# Autodesk Inventor assembly: MaquinaDeCorte
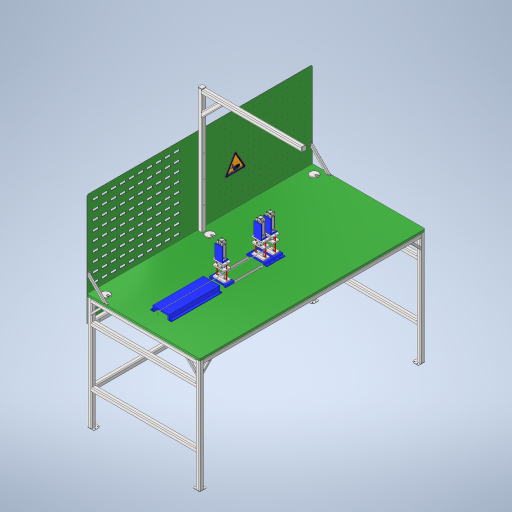
[picture p0: Inventor's stored thumbnail of the model, 512x512]
Saved by Autodesk Inventor 2023 (Build 270158000, 158)
## iProperties
Created: 2023-04-07
Part Number: MaquinaDeCorte
Document SubType Name: Assembly
Designer: Lenovo
Author: Lenovo
## Documents named in this file (35)
- D:\Esdek\Gemelo Digital\Corte de Tubos\MaquinaDeCorte.iam
- D:\Esdek\Gemelo Digital\Corte de Tubos\CADimportados\PistónElectromecánico\1470706 EPCO-25-300-3P-ST-E---(0).iam
- D:\Esdek\Gemelo Digital\Corte de Tubos\SoporteElectromecánico.ipt
- D:\Esdek\Gemelo Digital\Corte de Tubos\CADimportados\Main Table Assembly.ipt
- D:\Esdek\Gemelo Digital\Corte de Tubos\CADimportados\PistónHidráulico\163321 DNC-32-50-PPV---(asm_0).iam
- D:\Esdek\Gemelo Digital\Corte de Tubos\SoporteHidráhulicos.ipt
- D:\Esdek\Gemelo Digital\Corte de Tubos\PlacaSuperiorHidráulicos.ipt
- D:\Esdek\Gemelo Digital\Corte de Tubos\CodoHidráulicos.ipt
- D:\Esdek\Gemelo Digital\Corte de Tubos\PlacaMediaHidráulicos.ipt
- D:\Esdek\Gemelo Digital\Corte de Tubos\Cuchilla.ipt
- D:\Esdek\Gemelo Digital\Corte de Tubos\PlacaBaseHidráulicos.ipt
- D:\Esdek\Gemelo Digital\Corte de Tubos\BaseCuchilla.ipt
- D:\Esdek\Gemelo Digital\Corte de Tubos\CADimportados\Knutec.de - Warning, Crushing of hands, according ISO EN DIN 7010_200.ipt
- D:\Esdek\Gemelo Digital\Corte de Tubos\CADimportados\PistónHidráulico\163321 DNC-32-50-PPV---(asm_0)_CPY.iam
- D:\Esdek\Gemelo Digital\Corte de Tubos\SoporteHidráhulicos_CPY.ipt
- D:\Esdek\Gemelo Digital\Corte de Tubos\PlacaSuperiorHidráulicos_CPY.ipt
- D:\Esdek\Gemelo Digital\Corte de Tubos\CodoHidráulicos_CPY.ipt
- D:\Esdek\Gemelo Digital\Corte de Tubos\PlacaMediaHidráulicos_CPY.ipt
- D:\Esdek\Gemelo Digital\Corte de Tubos\PlacaBaseHidráulicos_CPY.ipt
- D:\Esdek\Gemelo Digital\Corte de Tubos\SoporteTubosInferior.ipt
- D:\Esdek\Gemelo Digital\Corte de Tubos\SoporteTubosSuperior.ipt
- D:\Esdek\Gemelo Digital\Corte de Tubos\CADimportados\PistónHidráulico\163321 DNC-32-50-PPV---(asm_0)_CPY_CPY.iam
- D:\Esdek\Gemelo Digital\Corte de Tubos\SoporteHidráhulicos_CPY_CPY.ipt
- D:\Esdek\Gemelo Digital\Corte de Tubos\PlacaSuperiorHidráulicos_CPY_CPY.ipt
- D:\Esdek\Gemelo Digital\Corte de Tubos\CodoHidráulicos_CPY_CPY.ipt
- D:\Esdek\Gemelo Digital\Corte de Tubos\PlacaMediaHidráulicos_CPY_CPY.ipt
- D:\Esdek\Gemelo Digital\Corte de Tubos\PlacaBaseHidráulicos_CPY_CPY.ipt
- D:\Esdek\Gemelo Digital\Corte de Tubos\SoporteTubosInferior_CPY.ipt
- D:\Esdek\Gemelo Digital\Corte de Tubos\SoporteTubosSuperior_CPY.ipt
- D:\Esdek\Gemelo Digital\Corte de Tubos\AcopleActuadorCarro.ipt
- D:\Esdek\Gemelo Digital\Corte de Tubos\CarroSuperior.ipt
- D:\Esdek\Gemelo Digital\Corte de Tubos\CarroFijoSuperior.ipt
- D:\Esdek\Gemelo Digital\Corte de Tubos\Sujetador.ipt
- D:\Esdek\Gemelo Digital\Corte de Tubos\SoporteMaterial.ipt
- D:\Esdek\Gemelo Digital\Corte de Tubos\Material.ipt
## Components (41 placed, 34 different names)
1. 1470706 EPCO-25-300-3P-ST-E---(0):1 [sub-assembly] — Mate:30, Mate:31, Mate:32, Mate:33, Mate:34
2. Main Table Assembly:1 — Mate:25, Angle:1, Mate:26, Mate:27, Mate:28, Mate:29, Mate:87, Mate:88, Mate:89, Mate:93, Mate:94, Mate:95, Mate:111, Mate:112, Mate:113
3. 163321 DNC-32-50-PPV---(asm_0):1 [sub-assembly] — Mate:4, Mate:5, Mate:6, Mate:12
4. SoporteHidráhulicos:1 — Mate:4, Mate:5, Mate:6, Mate:7, Mate:8, Mate:9
5. PlacaSuperiorHidráulicos:1 — Mate:7, Mate:8, Mate:9, Mate:10, Mate:11, Mate:24, Mate:107, Mate:108, Mate:109, Mate:110
6. CodoHidráulicos:1 — Mate:10, Mate:11, Mate:12, Mate:13, Mate:14, Mate:15
7. PlacaMediaHidráulicos:1 — Mate:13, Mate:14, Mate:15, Mate:16, Mate:17, Mate:18, Mate:22, Mate:23
8. Cuchilla:1 — Mate:16, Mate:17, Mate:18
9. PlacaBaseHidráulicos:1 — Mate:19, Mate:20, Mate:21, Mate:22, Mate:23, Mate:96, Mate:97, Mate:98
10. BaseCuchilla:1 — Mate:19, Mate:20, Mate:21, Mate:24, Mate:115
11. Knutec.de - Warning, Crushing of hands, according ISO EN DIN 7010_200:1 — Mate:25, Angle:1, Mate:26
12. SoporteElectromecánico:1 — Mate:27, Mate:28, Mate:29, Mate:30, Mate:31, Mate:32, Angle:2
13. CodoHidráulicos:2 — Mate:33, Mate:34, Angle:2, Mate:78, Mate:79, Mate:80
14. 163321 DNC-32-50-PPV---(asm_0)_CPY:1 [sub-assembly] — Mate:36, Mate:37, Mate:38, Mate:42
15. SoporteHidráhulicos_CPY:1 — Mate:36, Mate:37, Mate:38, Mate:39, Mate:40, Mate:41
16. PlacaSuperiorHidráulicos_CPY:1 — Mate:39, Mate:40, Mate:41, Mate:43, Mate:44, Mate:50, Mate:104, Mate:105, Mate:106
17. CodoHidráulicos_CPY:1 — Mate:42, Mate:43, Mate:44, Mate:45, Mate:46, Mate:47
18. PlacaMediaHidráulicos_CPY:1 — Mate:45, Mate:46, Mate:47, Mate:48, Mate:49, Mate:54, Mate:55, Mate:56, Mate:103
19. PlacaBaseHidráulicos_CPY:1 — Mate:48, Mate:49, Mate:50, Mate:51, Mate:52, Mate:53, Mate:90, Mate:91, Mate:92
20. SoporteTubosInferior:1 — Mate:51, Mate:52, Mate:53
21. SoporteTubosSuperior:1 — Mate:54, Mate:55, Mate:56
22. 163321 DNC-32-50-PPV---(asm_0)_CPY_CPY:1 [sub-assembly] — Mate:57, Mate:58, Mate:59, Mate:65
23. SoporteHidráhulicos_CPY_CPY:1 — Mate:57, Mate:58, Mate:59, Mate:60, Mate:61, Mate:62
24. PlacaSuperiorHidráulicos_CPY_CPY:1 — Mate:60, Mate:61, Mate:62, Mate:63, Mate:64, Mate:69, Mate:99, Mate:100, Mate:102
25. CodoHidráulicos_CPY_CPY:1 — Mate:63, Mate:64, Mate:65, Mate:66, Mate:67, Mate:68
26. PlacaMediaHidráulicos_CPY_CPY:1 — Mate:66, Mate:67, Mate:68, Mate:70, Mate:71, Mate:75, Mate:76, Mate:77, Mate:101
27. PlacaBaseHidráulicos_CPY_CPY:1 — Mate:69, Mate:70, Mate:71, Mate:72, Mate:73, Mate:74, Mate:84, Mate:85, Mate:86
28. SoporteTubosInferior_CPY:1 — Mate:72, Mate:73, Mate:74
29. SoporteTubosSuperior_CPY:1 — Mate:75, Mate:76, Mate:77
30. AcopleActuadorCarro:1 — Mate:78, Mate:79, Mate:80, Mate:81, Mate:82, Mate:83
31. CarroSuperior:1 — Mate:81, Mate:82, Mate:83, Mate:84, Mate:85, Mate:86
32. CarroFijoSuperior:1 — Mate:87, Mate:88, Mate:89, Mate:90, Mate:91, Mate:92
33. CarroFijoSuperior:2 — Mate:93, Mate:94, Mate:95, Mate:96, Mate:97, Mate:98
34. Sujetador:1 — Mate:99, Mate:100
35. Sujetador:2 — Mate:101, Mate:102
36. Sujetador:3 — Mate:103, Mate:104
37. Sujetador:4 — Mate:107, Mate:108
38. Sujetador:5 — Mate:109, Mate:110
39. Sujetador:6 — Mate:105, Mate:106
40. SoporteMaterial:1 — Mate:111, Mate:112, Mate:113, Mate:114
41. Material:1 — Mate:114, Mate:115
## Relationships (113: Mate 111, Angle 2)
- Mate:4: 163321 DNC-32-50-PPV---(asm_0):1 ↔ SoporteHidráhulicos:1
- Mate:5: 163321 DNC-32-50-PPV---(asm_0):1 ↔ SoporteHidráhulicos:1
- Mate:6: 163321 DNC-32-50-PPV---(asm_0):1 ↔ SoporteHidráhulicos:1
- Mate:7: SoporteHidráhulicos:1 ↔ PlacaSuperiorHidráulicos:1
- Mate:8: SoporteHidráhulicos:1 ↔ PlacaSuperiorHidráulicos:1
- Mate:9: SoporteHidráhulicos:1 ↔ PlacaSuperiorHidráulicos:1
- Mate:10: PlacaSuperiorHidráulicos:1 ↔ CodoHidráulicos:1
- Mate:11: PlacaSuperiorHidráulicos:1 ↔ CodoHidráulicos:1
- Mate:12: 163321 DNC-32-50-PPV---(asm_0):1 ↔ CodoHidráulicos:1
- Mate:13: CodoHidráulicos:1 ↔ PlacaMediaHidráulicos:1
- Mate:14: CodoHidráulicos:1 ↔ PlacaMediaHidráulicos:1
- Mate:15: CodoHidráulicos:1 ↔ PlacaMediaHidráulicos:1
- Mate:16: PlacaMediaHidráulicos:1 ↔ Cuchilla:1
- Mate:17: PlacaMediaHidráulicos:1 ↔ Cuchilla:1
- Mate:18: PlacaMediaHidráulicos:1 ↔ Cuchilla:1
- Mate:19: PlacaBaseHidráulicos:1 ↔ BaseCuchilla:1
- Mate:20: PlacaBaseHidráulicos:1 ↔ BaseCuchilla:1
- Mate:21: PlacaBaseHidráulicos:1 ↔ BaseCuchilla:1
- Mate:22: PlacaMediaHidráulicos:1 ↔ PlacaBaseHidráulicos:1
- Mate:23: PlacaMediaHidráulicos:1 ↔ PlacaBaseHidráulicos:1
- Mate:24 (115.5 mm): PlacaSuperiorHidráulicos:1 ↔ BaseCuchilla:1
- Mate:25: Main Table Assembly:1 ↔ Knutec.de - Warning, Crushing of hands, according ISO EN DIN 7010_200:1
- Angle:1 (180 deg): Main Table Assembly:1 ↔ Knutec.de - Warning, Crushing of hands, according ISO EN DIN 7010_200:1
- Mate:26: Main Table Assembly:1 ↔ Knutec.de - Warning, Crushing of hands, according ISO EN DIN 7010_200:1
- Mate:27: Main Table Assembly:1 ↔ SoporteElectromecánico:1
- Mate:28: Main Table Assembly:1 ↔ SoporteElectromecánico:1
- Mate:29: Main Table Assembly:1 ↔ SoporteElectromecánico:1
- Mate:30: 1470706 EPCO-25-300-3P-ST-E---(0):1 ↔ SoporteElectromecánico:1
- Mate:31: 1470706 EPCO-25-300-3P-ST-E---(0):1 ↔ SoporteElectromecánico:1
- Mate:32: 1470706 EPCO-25-300-3P-ST-E---(0):1 ↔ SoporteElectromecánico:1
- Mate:33: 1470706 EPCO-25-300-3P-ST-E---(0):1 ↔ CodoHidráulicos:2
- Mate:34: 1470706 EPCO-25-300-3P-ST-E---(0):1 ↔ CodoHidráulicos:2
- Angle:2 (0 deg): SoporteElectromecánico:1 ↔ CodoHidráulicos:2
- Mate:36: 163321 DNC-32-50-PPV---(asm_0)_CPY:1 ↔ SoporteHidráhulicos_CPY:1
- Mate:37: 163321 DNC-32-50-PPV---(asm_0)_CPY:1 ↔ SoporteHidráhulicos_CPY:1
- Mate:38: 163321 DNC-32-50-PPV---(asm_0)_CPY:1 ↔ SoporteHidráhulicos_CPY:1
- Mate:39: SoporteHidráhulicos_CPY:1 ↔ PlacaSuperiorHidráulicos_CPY:1
- Mate:40: SoporteHidráhulicos_CPY:1 ↔ PlacaSuperiorHidráulicos_CPY:1
- Mate:41: SoporteHidráhulicos_CPY:1 ↔ PlacaSuperiorHidráulicos_CPY:1
- Mate:42: 163321 DNC-32-50-PPV---(asm_0)_CPY:1 ↔ CodoHidráulicos_CPY:1
- Mate:43: PlacaSuperiorHidráulicos_CPY:1 ↔ CodoHidráulicos_CPY:1
- Mate:44: PlacaSuperiorHidráulicos_CPY:1 ↔ CodoHidráulicos_CPY:1
- Mate:45: CodoHidráulicos_CPY:1 ↔ PlacaMediaHidráulicos_CPY:1
- Mate:46: CodoHidráulicos_CPY:1 ↔ PlacaMediaHidráulicos_CPY:1
- Mate:47: CodoHidráulicos_CPY:1 ↔ PlacaMediaHidráulicos_CPY:1
- Mate:48: PlacaMediaHidráulicos_CPY:1 ↔ PlacaBaseHidráulicos_CPY:1
- Mate:49: PlacaMediaHidráulicos_CPY:1 ↔ PlacaBaseHidráulicos_CPY:1
- Mate:50 (125.5 mm): PlacaSuperiorHidráulicos_CPY:1 ↔ PlacaBaseHidráulicos_CPY:1
- Mate:51: PlacaBaseHidráulicos_CPY:1 ↔ SoporteTubosInferior:1
- Mate:52: PlacaBaseHidráulicos_CPY:1 ↔ SoporteTubosInferior:1
- Mate:53: PlacaBaseHidráulicos_CPY:1 ↔ SoporteTubosInferior:1
- Mate:54: PlacaMediaHidráulicos_CPY:1 ↔ SoporteTubosSuperior:1
- Mate:55: PlacaMediaHidráulicos_CPY:1 ↔ SoporteTubosSuperior:1
- Mate:56: PlacaMediaHidráulicos_CPY:1 ↔ SoporteTubosSuperior:1
- Mate:57: 163321 DNC-32-50-PPV---(asm_0)_CPY_CPY:1 ↔ SoporteHidráhulicos_CPY_CPY:1
- Mate:58: 163321 DNC-32-50-PPV---(asm_0)_CPY_CPY:1 ↔ SoporteHidráhulicos_CPY_CPY:1
- Mate:59: 163321 DNC-32-50-PPV---(asm_0)_CPY_CPY:1 ↔ SoporteHidráhulicos_CPY_CPY:1
- Mate:60: SoporteHidráhulicos_CPY_CPY:1 ↔ PlacaSuperiorHidráulicos_CPY_CPY:1
- Mate:61: SoporteHidráhulicos_CPY_CPY:1 ↔ PlacaSuperiorHidráulicos_CPY_CPY:1
- Mate:62: SoporteHidráhulicos_CPY_CPY:1 ↔ PlacaSuperiorHidráulicos_CPY_CPY:1
- Mate:63: PlacaSuperiorHidráulicos_CPY_CPY:1 ↔ CodoHidráulicos_CPY_CPY:1
- Mate:64: PlacaSuperiorHidráulicos_CPY_CPY:1 ↔ CodoHidráulicos_CPY_CPY:1
- Mate:65: 163321 DNC-32-50-PPV---(asm_0)_CPY_CPY:1 ↔ CodoHidráulicos_CPY_CPY:1
- Mate:66: CodoHidráulicos_CPY_CPY:1 ↔ PlacaMediaHidráulicos_CPY_CPY:1
- Mate:67: CodoHidráulicos_CPY_CPY:1 ↔ PlacaMediaHidráulicos_CPY_CPY:1
- Mate:68: CodoHidráulicos_CPY_CPY:1 ↔ PlacaMediaHidráulicos_CPY_CPY:1
- Mate:69 (125.5 mm): PlacaSuperiorHidráulicos_CPY_CPY:1 ↔ PlacaBaseHidráulicos_CPY_CPY:1
- Mate:70: PlacaMediaHidráulicos_CPY_CPY:1 ↔ PlacaBaseHidráulicos_CPY_CPY:1
- Mate:71: PlacaMediaHidráulicos_CPY_CPY:1 ↔ PlacaBaseHidráulicos_CPY_CPY:1
- Mate:72: PlacaBaseHidráulicos_CPY_CPY:1 ↔ SoporteTubosInferior_CPY:1
- Mate:73: PlacaBaseHidráulicos_CPY_CPY:1 ↔ SoporteTubosInferior_CPY:1
- Mate:74: PlacaBaseHidráulicos_CPY_CPY:1 ↔ SoporteTubosInferior_CPY:1
- Mate:75: PlacaMediaHidráulicos_CPY_CPY:1 ↔ SoporteTubosSuperior_CPY:1
- Mate:76: PlacaMediaHidráulicos_CPY_CPY:1 ↔ SoporteTubosSuperior_CPY:1
- Mate:77: PlacaMediaHidráulicos_CPY_CPY:1 ↔ SoporteTubosSuperior_CPY:1
- Mate:78: CodoHidráulicos:2 ↔ AcopleActuadorCarro:1
- Mate:79: CodoHidráulicos:2 ↔ AcopleActuadorCarro:1
- Mate:80: CodoHidráulicos:2 ↔ AcopleActuadorCarro:1
- Mate:81: AcopleActuadorCarro:1 ↔ CarroSuperior:1
- Mate:82: AcopleActuadorCarro:1 ↔ CarroSuperior:1
- Mate:83: AcopleActuadorCarro:1 ↔ CarroSuperior:1
- Mate:84: PlacaBaseHidráulicos_CPY_CPY:1 ↔ CarroSuperior:1
- Mate:85: PlacaBaseHidráulicos_CPY_CPY:1 ↔ CarroSuperior:1
- Mate:86: PlacaBaseHidráulicos_CPY_CPY:1 ↔ CarroSuperior:1
- Mate:87: Main Table Assembly:1 ↔ CarroFijoSuperior:1
- Mate:88: Main Table Assembly:1 ↔ CarroFijoSuperior:1
- Mate:89: Main Table Assembly:1 ↔ CarroFijoSuperior:1
- Mate:90: PlacaBaseHidráulicos_CPY:1 ↔ CarroFijoSuperior:1
- Mate:91: PlacaBaseHidráulicos_CPY:1 ↔ CarroFijoSuperior:1
- Mate:92: PlacaBaseHidráulicos_CPY:1 ↔ CarroFijoSuperior:1
- Mate:93: Main Table Assembly:1 ↔ CarroFijoSuperior:2
- Mate:94: Main Table Assembly:1 ↔ CarroFijoSuperior:2
- Mate:95: Main Table Assembly:1 ↔ CarroFijoSuperior:2
- Mate:96: PlacaBaseHidráulicos:1 ↔ CarroFijoSuperior:2
- Mate:97: PlacaBaseHidráulicos:1 ↔ CarroFijoSuperior:2
- Mate:98: PlacaBaseHidráulicos:1 ↔ CarroFijoSuperior:2
- Mate:99: PlacaSuperiorHidráulicos_CPY_CPY:1 ↔ Sujetador:1
- Mate:100: PlacaSuperiorHidráulicos_CPY_CPY:1 ↔ Sujetador:1
- Mate:101: PlacaMediaHidráulicos_CPY_CPY:1 ↔ Sujetador:2
- Mate:102: PlacaSuperiorHidráulicos_CPY_CPY:1 ↔ Sujetador:2
- Mate:103: PlacaMediaHidráulicos_CPY:1 ↔ Sujetador:3
- Mate:104: PlacaSuperiorHidráulicos_CPY:1 ↔ Sujetador:3
- Mate:105: PlacaSuperiorHidráulicos_CPY:1 ↔ Sujetador:6
- Mate:106: PlacaSuperiorHidráulicos_CPY:1 ↔ Sujetador:6
- Mate:107: PlacaSuperiorHidráulicos:1 ↔ Sujetador:4
- Mate:108: PlacaSuperiorHidráulicos:1 ↔ Sujetador:4
- Mate:109: PlacaSuperiorHidráulicos:1 ↔ Sujetador:5
- Mate:110: PlacaSuperiorHidráulicos:1 ↔ Sujetador:5
- Mate:111: Main Table Assembly:1 ↔ SoporteMaterial:1
- Mate:112: Main Table Assembly:1 ↔ SoporteMaterial:1
- Mate:113: Main Table Assembly:1 ↔ SoporteMaterial:1
- Mate:114: SoporteMaterial:1 ↔ Material:1
- Mate:115 (5 mm): BaseCuchilla:1 ↔ Material:1
